# Autodesk Inventor assembly: yaw roll propuesta
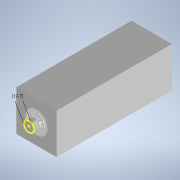
[picture p0: Inventor's stored thumbnail of the model, 180x180]
Saved by Autodesk Inventor 2020.3 (Build 243373000, 373)
## iProperties
Created: 2021-01-22
Part Number: yaw roll propuesta
Document SubType Name: Assembly
Designer: Yu Jinyu
Author: Yu Jinyu
## Documents named in this file (4)
- C:\Users\Yu Jinyu\OneDrive\Escritorio\Yaw Roll Nuevo\yaw roll propuesta.iam
- C:\Users\Yu Jinyu\OneDrive\Escritorio\Yaw Roll Nuevo\Motor Banebot.iam
- C:\Users\Yu Jinyu\OneDrive\Escritorio\Yaw Roll Nuevo\banebot soporte.ipt
- C:\Users\Yu Jinyu\OneDrive\Escritorio\Yaw Roll Nuevo\rodamientov2.ipt
## Components (3 placed, 3 different names)
1. Motor Banebot:1 [sub-assembly] — Insert:2
2. banebot soporte:1 — Insert:1
3. rodamientov2:1 — Insert:1, Insert:2
## Relationships (2: Insert 2)
- Insert:1 (-8 mm): banebot soporte:1 ↔ rodamientov2:1
- Insert:2 (70 mm): Motor Banebot:1 ↔ rodamientov2:1
